# Autodesk Inventor assembly: EX_Assembly
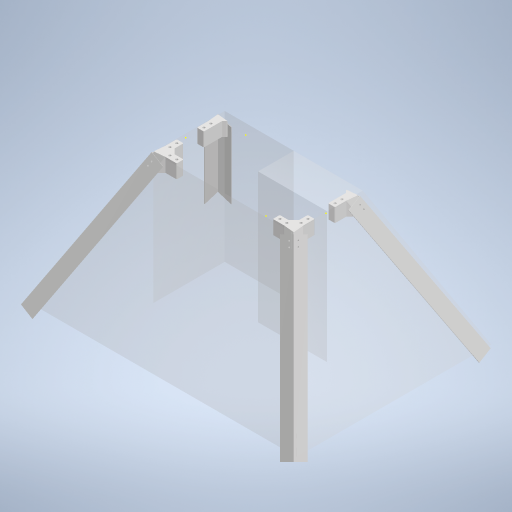
[picture p0: Inventor's stored thumbnail of the model, 512x512]
Saved by Autodesk Inventor 2024.3 (Build 283343000, 343)
## iProperties
Created: 2025-11-25
Part Number: EX_Assembly
Document SubType Name: Assembly
Designer: 佐藤智貴
Author: 佐藤智貴
## Documents named in this file (6)
- C:\Users\佐藤智貴\OneDrive - Chiba Institute of Technology\ドキュメント\Inventor\Biped_Robot2\EX_Assembly.iam
- C:\Users\佐藤智貴\OneDrive - Chiba Institute of Technology\ドキュメント\Inventor\Biped_Robot2\AA30306.ipt
- C:\Users\佐藤智貴\OneDrive - Chiba Institute of Technology\ドキュメント\Inventor\Biped_Robot2\EX-L-Connect-Front.ipt
- C:\Users\佐藤智貴\OneDrive - Chiba Institute of Technology\ドキュメント\Inventor\Biped_Robot2\EX-L-Connect-Back-Right.ipt
- C:\Users\佐藤智貴\OneDrive - Chiba Institute of Technology\ドキュメント\Inventor\Biped_Robot2\EX-L-Connect-Back-Left.ipt
- C:\Users\佐藤智貴\OneDrive - Chiba Institute of Technology\ドキュメント\Inventor\Biped_Robot2\PPsheet_500-300.ipt
## Components (9 placed, 5 different names)
1. AA30306:5 — 挿入:13, 挿入:14
2. AA30306:6 — 挿入:11, 挿入:12
3. AA30306:7 — 挿入:7, 挿入:8
4. AA30306:8 — 挿入:3, 挿入:4
5. EX-L-Connect-Front:1 — 挿入:11, 挿入:12
6. EX-L-Connect-Front:2 — 挿入:13, 挿入:14
7. EX-L-Connect-Back-Right:1 — 挿入:3, 挿入:4
8. EX-L-Connect-Back-Left:1 — 挿入:7, 挿入:8
9. PPsheet_500-300:1
## Relationships (8: Insert 8)
- 挿入:3 [Insert]: AA30306:8 ↔ EX-L-Connect-Back-Right:1
- 挿入:4 [Insert]: AA30306:8 ↔ EX-L-Connect-Back-Right:1
- 挿入:7 [Insert]: AA30306:7 ↔ EX-L-Connect-Back-Left:1
- 挿入:8 [Insert]: AA30306:7 ↔ EX-L-Connect-Back-Left:1
- 挿入:11 [Insert]: AA30306:6 ↔ EX-L-Connect-Front:1
- 挿入:12 [Insert]: AA30306:6 ↔ EX-L-Connect-Front:1
- 挿入:13 [Insert]: AA30306:5 ↔ EX-L-Connect-Front:2
- 挿入:14 [Insert]: AA30306:5 ↔ EX-L-Connect-Front:2
